# Autodesk Inventor assembly: SliderRight
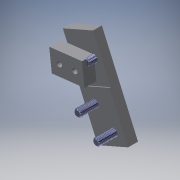
[picture p0: Inventor's stored thumbnail of the model, 180x180]
Saved by Autodesk Inventor 2019 (Build 230136000, 136)
## iProperties
Created: 2019-09-28
Part Number: SliderRight
Document SubType Name: Assembly
Designer: james
Author: james
## Documents named in this file (5)
- F:\JimsDesign\Jims2020FTC\SliderRight.iam
- F:\JimsDesign\Jims2020FTC\SliderBlock.ipt
- F:\JimsDesign\Jims2020FTC\SidePlateRight.ipt
- F:\JimsDesign\Library\McMaster\Screws\91771A196_18-8 SS FLAT HEAD PHILLIPS MACHINE SCREW.ipt
- F:\JimsDesign\Library\McMaster\Screws\91771A192_18-8 SS FLAT HEAD PHILLIPS MACHINE SCREW.ipt
## Components (6 placed, 4 different names)
1. SidePlateRight:1 — Mate:1, Mate:6, Mate:7, Flush:5, Flush:6, Flush:7, Flush:8, Mate:8, Mate:9
2. SliderBlock:1 — Mate:1
3. 91771A196_18-8 SS FLAT HEAD PHILLIPS MACHINE SCREW:3 — Flush:8, Mate:8
4. 91771A196_18-8 SS FLAT HEAD PHILLIPS MACHINE SCREW:4 — Flush:7, Mate:9
5. 91771A192_18-8 SS FLAT HEAD PHILLIPS MACHINE SCREW:1 — Mate:6, Flush:6
6. 91771A192_18-8 SS FLAT HEAD PHILLIPS MACHINE SCREW:2 — Mate:7, Flush:5
## Relationships (9: Mate 5, Flush 4)
- Mate:1: SidePlateRight:1 ↔ SliderBlock:1
- Mate:6: SidePlateRight:1 ↔ 91771A192_18-8 SS FLAT HEAD PHILLIPS MACHINE SCREW:1
- Mate:7: SidePlateRight:1 ↔ 91771A192_18-8 SS FLAT HEAD PHILLIPS MACHINE SCREW:2
- Flush:5: SidePlateRight:1 ↔ 91771A192_18-8 SS FLAT HEAD PHILLIPS MACHINE SCREW:2
- Flush:6: SidePlateRight:1 ↔ 91771A192_18-8 SS FLAT HEAD PHILLIPS MACHINE SCREW:1
- Flush:7: SidePlateRight:1 ↔ 91771A196_18-8 SS FLAT HEAD PHILLIPS MACHINE SCREW:4
- Flush:8: SidePlateRight:1 ↔ 91771A196_18-8 SS FLAT HEAD PHILLIPS MACHINE SCREW:3
- Mate:8: SidePlateRight:1 ↔ 91771A196_18-8 SS FLAT HEAD PHILLIPS MACHINE SCREW:3
- Mate:9: SidePlateRight:1 ↔ 91771A196_18-8 SS FLAT HEAD PHILLIPS MACHINE SCREW:4
